# Autodesk Inventor assembly: sensorHolder
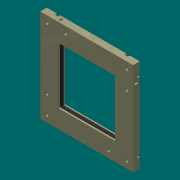
[picture p0: Inventor's stored thumbnail of the model, 180x180]
Saved by Autodesk Inventor 2016 (Build 200138000, 138)
## iProperties
Created: 2015-10-19
Part Number: sensorHolder
Document SubType Name: Assembly
Designer: Sawaiz
Author: Sawaiz
## Documents named in this file (5)
- C:\Users\Sawaiz\OneDrive\projects\modularRICH\frame\sensorHolder.iam
- C:\Users\Sawaiz\OneDrive\projects\modularRICH\frame\sensorORing.ipt
- C:\Users\Sawaiz\OneDrive\projects\modularRICH\frame\sensorHolder.ipt
- C:\Users\Sawaiz\OneDrive\projects\modularRICH\frame\sensorHolderFlushORing.ipt
- C:\Users\Sawaiz\OneDrive\projects\modularRICH\modularRICH.xlsx
## Components (6 placed, 3 different names)
1. sensorORing:1 — Mate:4, Mate:5, Mate:9
2. sensorHolder:1 — Flush:3, Mate:4, Mate:5, Flush:4, Mate:7, Mate:8, Flush:6, Mate:10, Mate:12
3. sensorHolder:2 — Flush:1, Mate:8, Flush:6, Mate:9
4. sensorHolder:3 — Flush:2, Flush:3, Flush:4, Flush:5, Mate:6, Mate:7, Mate:11
5. sensorHolder:4 — Flush:1, Flush:2, Flush:5, Mate:6
6. sensorHolderFlushORing:1 — Mate:10, Mate:11, Mate:12
## Relationships (15: Mate 9, Flush 6)
- Flush:1: sensorHolder:2 ↔ sensorHolder:4
- Flush:2: sensorHolder:3 ↔ sensorHolder:4
- Flush:3: sensorHolder:1 ↔ sensorHolder:3
- Mate:4: sensorORing:1 ↔ sensorHolder:1
- Mate:5: sensorORing:1 ↔ sensorHolder:1
- Flush:4: sensorHolder:1 ↔ sensorHolder:3
- Flush:5: sensorHolder:3 ↔ sensorHolder:4
- Mate:6: sensorHolder:3 ↔ sensorHolder:4
- Mate:7: sensorHolder:1 ↔ sensorHolder:3
- Mate:8: sensorHolder:1 ↔ sensorHolder:2
- Flush:6: sensorHolder:1 ↔ sensorHolder:2
- Mate:9: sensorORing:1 ↔ sensorHolder:2
- Mate:10: sensorHolder:1 ↔ sensorHolderFlushORing:1
- Mate:11: sensorHolder:3 ↔ sensorHolderFlushORing:1
- Mate:12: sensorHolder:1 ↔ sensorHolderFlushORing:1
## Named parameters: acrylicThickness = 6.35 mm, aerogelThickness = 20 mm, height = 101.6 mm, width = 101.6 mm, depth = 101.6 mm, mirrorAngle = 5 deg, detectorWidth = 52 mm, detectorHeight = 52 mm, mirrorThickness = 3 mm, fresnelThickness = 0.1 mm, grooveDensity = 100, focalLength = 76.2 mm, ior = 1.49, centerThickness = 1.524 mm, fresnelAngle = 90 deg, fresnelEffectiveDiameter = 76.2 mm, mirrorSuppourtWidth = 38.1 mm, backGrooveBit = 4.8006 mm, sensorHolderWidth = 88.9 mm, sensorHolderHeight = 88.9 mm, sensorHolderSensorHeight = 53.975 mm, sensorHolderSensorWidth = 53.975 mm, sensorHolderORing = 3.175 mm, sensorHolderFlushORing = 3.175 mm, sensorHolderFlushORingID = 304.8 mm, oRingWidth = 3.175 mm, sensorHolderORingID = 203.2 mm, frontBackORingID = 419.1 mm, topBottomHorizontalMirrorGroove = 12.7 mm, backMirrorGroove = 6.35 mm, mirrorGroove = 19.05 mm, compressionPercent = 40, fresnelChamfer = 6.35 mm, mirrorGrooveFillet = 6.35 mm, mirrorGrooveDrill = 6.35 mm, mirrorGrooveMill = 3.175 mm, fresnelMirrorChamfer = 6.35 mm, detectorOpeningWidth = 76.2 mm, detectorOpeningHeight = 76.2 mm
